# Autodesk Inventor assembly: 机械手部件连接
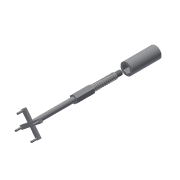
[picture p0: Inventor's stored thumbnail of the model, 180x180]
Saved by Autodesk Inventor 2016 (Build 200138000, 138)
## iProperties
Created: 2019-05-18
Part Number: 机械手部件连接
Material: 常规
Document SubType Name: Assembly
Designer: oldboy
Author: oldboy
## Documents named in this file (4)
- F:\folder\毕业设计\解魔方机器人\机械结构\机械手部件连接.iam
- F:\folder\毕业设计\解魔方机器人\机械结构\杆件.ipt
- F:\folder\毕业设计\解魔方机器人\机械结构\机械爪六角筒.ipt
- F:\folder\毕业设计\解魔方机器人\机械结构\机械手部件连接\设计加速器\压缩弹簧2.iam
## Components (3 placed, 3 different names)
1. 杆件:1 — 插入:1, 配合:2, 配合:3, 表面齐平:1
2. 机械爪六角筒:1 — 插入:1, 配合:2
3. 压缩弹簧:1 [sub-assembly] — 配合:3, 表面齐平:1
## Relationships (4: Mate 2, Insert 1, Flush 1)
- 插入:1 [Insert] (30 mm): 杆件:1 ↔ 机械爪六角筒:1
- 配合:2 [Mate]: 杆件:1 ↔ 机械爪六角筒:1
- 配合:3 [Mate]: 杆件:1 ↔ 压缩弹簧:1
- 表面齐平:1 [Flush]: 杆件:1 ↔ 压缩弹簧:1
